# Autodesk Inventor assembly: claws
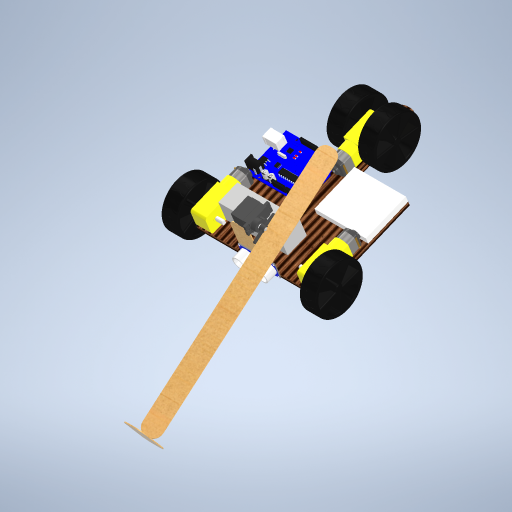
[picture p0: Inventor's stored thumbnail of the model, 512x512]
Saved by Autodesk Inventor 2023 (Build 270158000, 158)
## iProperties
Created: 2023-01-20
Part Number: claws
Document SubType Name: Assembly
Designer: kavya
Author: kavya
## Documents named in this file (11)
- C:\Users\kavya\OneDrive\Documents\OEC\claws.iam
- C:\Users\kavya\OneDrive\Documents\OEC\base.ipt
- C:\Users\kavya\OneDrive\Documents\OEC\wheel.ipt
- C:\Users\kavya\OneDrive\Documents\OEC\arduino-uno.snapshot.3\arduino uno.iam
- C:\Users\kavya\OneDrive\Documents\OEC\arduino-gear-motor-1.snapshot.4\Arduino Gear Motor.ipt
- C:\Users\kavya\OneDrive\Documents\OEC\hc-sr04-y-mg90s-1.snapshot.3\ensamble total\servo motor MG90S\ensamble.iam
- C:\Users\kavya\OneDrive\Documents\OEC\hc-sr04-y-mg90s-1.snapshot.3\ensamble total\PARTE 1.ipt
- C:\Users\kavya\OneDrive\Documents\OEC\popsicle stick.ipt
- C:\Users\kavya\OneDrive\Documents\OEC\popsicle stick - Copy.ipt
- C:\Users\kavya\OneDrive\Documents\OEC\board.ipt
- C:\Users\kavya\OneDrive\Documents\OEC\battery.ipt
## Components (16 placed, 10 different names)
1. base:1 — Mate:1, Mate:2, Flush:3, Mate:3, Flush:4, Flush:5, Flush:6, Mate:4, Mate:5, Flush:7, Flush:8, Flush:9, Flush:10, Mate:9, Mate:12, Flush:11, Flush:12, Mate:13, Flush:13, Flush:14, Mate:18
2. arduino uno:1 [sub-assembly] — Mate:12, Flush:11, Flush:12
3. Arduino Gear Motor:1 — Mate:1, Mate:2, Insert:5, Insert:6, Flush:9, Flush:10
4. Arduino Gear Motor:3 — Insert:3, Flush:3, Mate:3, Flush:4
5. wheel:2 — Insert:3
6. wheel:4 — Insert:6
7. Arduino Gear Motor:4 — Flush:5, Flush:6, Mate:4, Mate:19
8. wheel:6
9. ensamble:1 [sub-assembly] — Mate:10, Flush:15, Mate:16
10. PARTE 1:1 — Mate:5, Flush:7, Flush:8, Mate:15, Flush:16
11. popsicle stick:1 — Mate:16, Mate:17
12. wheel:7 — Insert:5
13. popsicle stick - Copy:1 — Mate:9, Mate:10, Flush:15, Mate:15, Flush:16
14. board:1 — Mate:13, Flush:13, Flush:14
15. popsicle stick - Copy:2 — Mate:17
16. battery:1 — Mate:18, Mate:19
## Relationships (32: Mate 14, Flush 14, Insert 4)
- Insert:3: Arduino Gear Motor:3 ↔ wheel:2
- [Insert]: Arduino Gear Motor:4 ↔ wheel:6
- Mate:1: base:1 ↔ Arduino Gear Motor:1
- Mate:2: base:1 ↔ Arduino Gear Motor:1
- Flush:3: base:1 ↔ Arduino Gear Motor:3
- Mate:3: base:1 ↔ Arduino Gear Motor:3
- Flush:4: base:1 ↔ Arduino Gear Motor:3
- Flush:5: base:1 ↔ Arduino Gear Motor:4
- Flush:6: base:1 ↔ Arduino Gear Motor:4
- Mate:4: base:1 ↔ Arduino Gear Motor:4
- Mate:5: base:1 ↔ PARTE 1:1
- Flush:7: base:1 ↔ PARTE 1:1
- Flush:8: base:1 ↔ PARTE 1:1
- Insert:5 (-7.112 mm): Arduino Gear Motor:1 ↔ wheel:7
- Insert:6 (-9.271 mm): Arduino Gear Motor:1 ↔ wheel:4
- Flush:9: base:1 ↔ Arduino Gear Motor:1
- Flush:10: base:1 ↔ Arduino Gear Motor:1
- Mate:9: base:1 ↔ popsicle stick - Copy:1
- Mate:10: ensamble:1 ↔ popsicle stick - Copy:1
- Mate:12: base:1 ↔ arduino uno:1
- Flush:11: base:1 ↔ arduino uno:1
- Flush:12: base:1 ↔ arduino uno:1
- Mate:13: base:1 ↔ board:1
- Flush:13: base:1 ↔ board:1
- Flush:14: base:1 ↔ board:1
- Flush:15: ensamble:1 ↔ popsicle stick - Copy:1
- Mate:15: PARTE 1:1 ↔ popsicle stick - Copy:1
- Flush:16: PARTE 1:1 ↔ popsicle stick - Copy:1
- Mate:16: ensamble:1 ↔ popsicle stick:1
- Mate:17: popsicle stick:1 ↔ popsicle stick - Copy:2
- Mate:18: base:1 ↔ battery:1
- Mate:19: Arduino Gear Motor:4 ↔ battery:1
## Named parameters: d3_d2 = 0 mm
